# Autodesk Inventor assembly: POM_T5_01
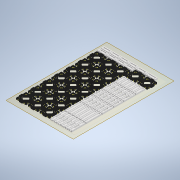
[picture p0: Inventor's stored thumbnail of the model, 180x180]
Saved by Autodesk Inventor 2022 (Build 260153000, 153)
## iProperties
Created: 2022-09-28
Part Number: POM_T5_01
Document SubType Name: Assembly
Designer: Masato
Author: Masato
## Documents named in this file (10)
- C:\Users\ヨコオリク\Documents\CITBrains\SUSTAINA-OP\Cam\POM_T5\POM_T5_01.iam
- C:\Users\ヨコオリク\Documents\CITBrains\SUSTAINA-OP\Cam\DisposableBoard.ipt
- C:\Users\ヨコオリク\Documents\CITBrains\SUSTAINA-OP\UpperBody\Arm\UpperArm_diagonal.ipt
- C:\Users\ヨコオリク\Documents\CITBrains\SUSTAINA-OP\OptionParts\DrillingJigs\BackLink_diagonal_Jig.ipt
- C:\Users\ヨコオリク\Documents\CITBrains\SUSTAINA-OP\OptionParts\DrillingJigs\Foot_root_block_Jig.ipt
- C:\Users\ヨコオリク\Documents\CITBrains\SUSTAINA-OP\OptionParts\DrillingJigs\FrontLink_diagonal_Jig.ipt
- C:\Users\ヨコオリク\Documents\CITBrains\SUSTAINA-OP\OptionParts\DrillingJigs\Leg_joint_yaw_frame_Jig.ipt
- C:\Users\ヨコオリク\Documents\CITBrains\SUSTAINA-OP\OptionParts\DrillingJigs\Trunk_lower_side_frame_Jig.ipt
- C:\Users\ヨコオリク\Documents\CITBrains\SUSTAINA-OP\OptionParts\DrillingJigs\UpperArm_diagonal_Jig.ipt
- C:\Users\ヨコオリク\Documents\CITBrains\SUSTAINA-OP\OptionParts\DrillingJigs\UpperBoby_horn_frame_Jig.ipt
## Components (70 placed, 9 different names)
1. DisposableBoard:1 — フラッシュ:1, フラッシュ:2, フラッシュ:3, フラッシュ:4, フラッシュ:5, フラッシュ:6, フラッシュ:7, フラッシュ:8
2. UpperArm_diagonal:1 — メイト:1, フラッシュ:5, フラッシュ:6
3. UpperArm_diagonal:2
4. UpperArm_diagonal:3 — メイト:9
5. UpperArm_diagonal:4
6. UpperArm_diagonal:5
7. UpperArm_diagonal:6 — メイト:11
8. UpperArm_diagonal:7
9. UpperArm_diagonal:8
10. UpperArm_diagonal:9
11. UpperArm_diagonal:10
12. UpperArm_diagonal:11
13. UpperArm_diagonal:12 — メイト:13
14. UpperArm_diagonal:13
15. UpperArm_diagonal:14
16. UpperArm_diagonal:15 — メイト:15
17. UpperArm_diagonal:16
18. UpperArm_diagonal:17
19. UpperArm_diagonal:18 — メイト:17
20. UpperArm_diagonal:19 — メイト:19
21. UpperArm_diagonal:20
22. UpperArm_diagonal:21 — メイト:21
23. Trunk_lower_side_frame_Jig:1 — メイト:7, フラッシュ:7, メイト:9, メイト:10
24. Trunk_lower_side_frame_Jig:2
25. Trunk_lower_side_frame_Jig:3
26. Trunk_lower_side_frame_Jig:4
27. Trunk_lower_side_frame_Jig:5
28. Trunk_lower_side_frame_Jig:6
29. FrontLink_diagonal_Jig:1 — メイト:3, メイト:10, メイト:11, メイト:12
30. FrontLink_diagonal_Jig:2
31. FrontLink_diagonal_Jig:3
32. FrontLink_diagonal_Jig:4
33. FrontLink_diagonal_Jig:5
34. FrontLink_diagonal_Jig:6
35. UpperBoby_horn_frame_Jig:1 — メイト:5, メイト:12, メイト:13, メイト:14
36. Leg_joint_yaw_frame_Jig:1 — メイト:8, メイト:14, メイト:15, メイト:16
37. UpperArm_diagonal_Jig:1 — メイト:6, メイト:16, メイト:17, メイト:18
38. BackLink_diagonal_Jig:1 — メイト:2, メイト:18
39. UpperBoby_horn_frame_Jig:2
40. Leg_joint_yaw_frame_Jig:2
41. UpperArm_diagonal_Jig:2
42. BackLink_diagonal_Jig:2 — メイト:22
43. UpperBoby_horn_frame_Jig:3
44. Leg_joint_yaw_frame_Jig:3
45. UpperArm_diagonal_Jig:3
46. BackLink_diagonal_Jig:3
47. UpperBoby_horn_frame_Jig:4
48. Leg_joint_yaw_frame_Jig:4
49. UpperArm_diagonal_Jig:4
50. BackLink_diagonal_Jig:4
51. UpperBoby_horn_frame_Jig:5
52. Leg_joint_yaw_frame_Jig:5
53. UpperArm_diagonal_Jig:5
54. BackLink_diagonal_Jig:5
55. UpperBoby_horn_frame_Jig:6
56. Leg_joint_yaw_frame_Jig:6
57. UpperArm_diagonal_Jig:6
58. BackLink_diagonal_Jig:6
59. Foot_root_block_Jig:1 — メイト:4, フラッシュ:8, メイト:19
60. Foot_root_block_Jig:2
61. Foot_root_block_Jig:3
62. Foot_root_block_Jig:4
63. Foot_root_block_Jig:5
64. Foot_root_block_Jig:6
65. Foot_root_block_Jig:7
66. Foot_root_block_Jig:8 — メイト:24
67. UpperArm_diagonal:22 — メイト:20, メイト:21, メイト:22, メイト:25
68. UpperArm_diagonal:23
69. BackLink_diagonal_Jig:7 — メイト:23, メイト:24, メイト:25
70. BackLink_diagonal_Jig:8
## Component patterns: (21 elements, first: UpperArm_diagonal:1), (6 elements, first: Trunk_lower_side_frame_Jig:1), (6 elements, first: FrontLink_diagonal_Jig:1), (6 elements, first: UpperBoby_horn_frame_Jig:1 + Leg_joint_yaw_frame_Jig:1 + UpperArm_diagonal_Jig:1 + BackLink_diagonal_Jig:1), (8 elements, first: Foot_root_block_Jig:1), (2 elements, first: UpperArm_diagonal:22), (2 elements, first: BackLink_diagonal_Jig:7)
## Relationships (33: Mate 25, Flush 8)
- フラッシュ:1 [Flush]: DisposableBoard:1
- フラッシュ:2 [Flush]: DisposableBoard:1
- フラッシュ:3 [Flush]: DisposableBoard:1
- フラッシュ:4 [Flush]: DisposableBoard:1
- メイト:1 [Mate]: UpperArm_diagonal:1
- メイト:2 [Mate]: BackLink_diagonal_Jig:1
- メイト:3 [Mate]: FrontLink_diagonal_Jig:1
- メイト:4 [Mate]: Foot_root_block_Jig:1
- メイト:5 [Mate]: UpperBoby_horn_frame_Jig:1
- メイト:6 [Mate]: UpperArm_diagonal_Jig:1
- メイト:7 [Mate]: Trunk_lower_side_frame_Jig:1
- メイト:8 [Mate]: Leg_joint_yaw_frame_Jig:1
- フラッシュ:5 [Flush] (2 mm): DisposableBoard:1 ↔ UpperArm_diagonal:1
- フラッシュ:6 [Flush] (2 mm): DisposableBoard:1 ↔ UpperArm_diagonal:1
- フラッシュ:7 [Flush] (2 mm): DisposableBoard:1 ↔ Trunk_lower_side_frame_Jig:1
- メイト:9 [Mate] (2.1 mm): UpperArm_diagonal:3 ↔ Trunk_lower_side_frame_Jig:1
- メイト:10 [Mate] (2.1 mm): Trunk_lower_side_frame_Jig:1 ↔ FrontLink_diagonal_Jig:1
- メイト:11 [Mate] (2.1 mm): UpperArm_diagonal:6 ↔ FrontLink_diagonal_Jig:1
- メイト:12 [Mate] (2.1 mm): FrontLink_diagonal_Jig:1 ↔ UpperBoby_horn_frame_Jig:1
- メイト:13 [Mate] (2.1 mm): UpperArm_diagonal:12 ↔ UpperBoby_horn_frame_Jig:1
- メイト:14 [Mate] (2.1 mm): UpperBoby_horn_frame_Jig:1 ↔ Leg_joint_yaw_frame_Jig:1
- メイト:15 [Mate] (2.1 mm): UpperArm_diagonal:15 ↔ Leg_joint_yaw_frame_Jig:1
- メイト:16 [Mate] (2.1 mm): Leg_joint_yaw_frame_Jig:1 ↔ UpperArm_diagonal_Jig:1
- メイト:17 [Mate] (2.1 mm): UpperArm_diagonal:18 ↔ UpperArm_diagonal_Jig:1
- メイト:18 [Mate] (2.1 mm): UpperArm_diagonal_Jig:1 ↔ BackLink_diagonal_Jig:1
- フラッシュ:8 [Flush] (2 mm): DisposableBoard:1 ↔ Foot_root_block_Jig:1
- メイト:19 [Mate] (2.1 mm): UpperArm_diagonal:19 ↔ Foot_root_block_Jig:1
- メイト:20 [Mate]: UpperArm_diagonal:22
- メイト:21 [Mate] (2.1 mm): UpperArm_diagonal:21 ↔ UpperArm_diagonal:22
- メイト:22 [Mate] (2.1 mm): BackLink_diagonal_Jig:2 ↔ UpperArm_diagonal:22
- メイト:23 [Mate]: BackLink_diagonal_Jig:7
- メイト:24 [Mate] (2.1 mm): Foot_root_block_Jig:8 ↔ BackLink_diagonal_Jig:7
- メイト:25 [Mate] (2.1 mm): UpperArm_diagonal:22 ↔ BackLink_diagonal_Jig:7
